# Autodesk Inventor assembly: BoxWithCover
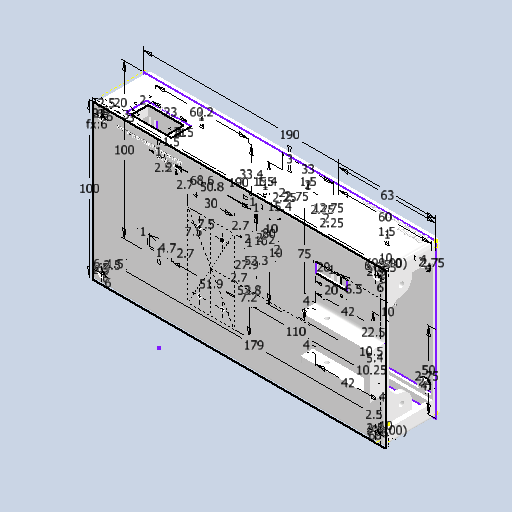
[picture p0: Inventor's stored thumbnail of the model, 512x512]
Saved by Autodesk Inventor 2023 (Build 270158000, 158)
## iProperties
Created: 2022-10-22
Part Number: BoxWithCover
Document SubType Name: Assembly
Designer: Miner
Author: Miner
## Documents named in this file (3)
- D:\AKFS\OneDrive - RMIT University\0. Main Research\139. Spectral Camera\GiTHub\3D Design and Parts\Enclosure with Cover.iam
- D:\AKFS\OneDrive - RMIT University\0. Main Research\139. Spectral Camera\3D parts\Box.ipt
- D:\AKFS\OneDrive - RMIT University\0. Main Research\139. Spectral Camera\3D parts\BoxCover.ipt
## Components (2 placed, 2 different names)
1. Box:1 — Rotational:1
2. BoxCover:1 — Rotational:1
## Relationships (1: RevoluteJoint 1)
- Rotational:1 [RevoluteJoint]: Box:1 ↔ BoxCover:1
